# Autodesk Inventor assembly: wheel with sprocket
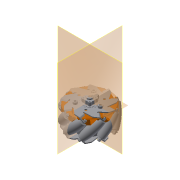
[picture p0: Inventor's stored thumbnail of the model, 180x180]
Saved by Autodesk Inventor 2018 (Build 220112000, 112)
## iProperties
Created: 2019-09-29
Part Number: wheel with sprocket
Document SubType Name: Assembly
Designer: ball
Author: ball
## Documents named in this file (3)
- C:\FTC\FTC8863CAD\2019 Robot\Mecanum Drive Train\wheel with sprocket.iam
- C:\FTC\FTC8863CAD\2019 Robot\Mecanum Drive Train\left wheel with clamping hub.iam
- C:\FTC\FTC8863CAD\Actobotics\615 parts\615102.ipt
## Components (2 placed, 2 different names)
1. left wheel with clamping hub:1 [sub-assembly] — Mate:1, Mate:2, Mate:3, Mate:4, Mate:5
2. 615102:1 — Mate:1, Mate:2, Mate:3
## Relationships (5: Mate 5)
- Mate:1: left wheel with clamping hub:1 ↔ 615102:1
- Mate:2: left wheel with clamping hub:1 ↔ 615102:1
- Mate:3 (2.54 mm): left wheel with clamping hub:1 ↔ 615102:1
- Mate:4: left wheel with clamping hub:1
- Mate:5: left wheel with clamping hub:1
